# Autodesk Inventor assembly: Estructura Lámina
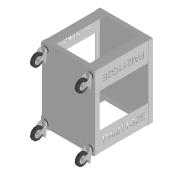
[picture p0: Inventor's stored thumbnail of the model, 180x180]
Saved by Autodesk Inventor 2021 (Build 250183000, 183)
## iProperties
Created: 2021-04-18
Part Number: Estructura Lámina
Document SubType Name: Assembly
Designer: carlo
Author: carlo
## Documents named in this file (4)
- C:\Users\carlo\Desktop\Concepto\Estructura laminas\Estructura Lámina.iam
- C:\Users\carlo\Desktop\Concepto\Estructura laminas\Laterales.ipt
- C:\Users\carlo\Desktop\Concepto\Estructura laminas\Tapa.ipt
- C:\Users\carlo\Desktop\Concepto\Estructura laminas\CASTER_WHEEL_FREE_Ø125mm.iam
## Components (10 placed, 3 different names)
1. Laterales:1 — Coincidencia:1, Coincidencia:2, Coincidencia:3
2. Tapa:1 — Coincidencia:1, Coincidencia:2, Coincidencia:3, Coincidencia:4, Coincidencia:5, Coincidencia:6, Coincidencia:7, Coincidencia:8, Coincidencia:9, Coincidencia:10, Coincidencia:11, Coincidencia:12
3. Laterales:2 — Coincidencia:7, Coincidencia:8, Coincidencia:9, Coincidencia:13, Coincidencia:14, Coincidencia:15
4. Laterales:3 — Coincidencia:10, Coincidencia:11, Coincidencia:12
5. Laterales:4 — Coincidencia:4, Coincidencia:5, Coincidencia:6
6. Tapa:2 — Coincidencia:13, Coincidencia:14, Coincidencia:15, Coincidencia:16, Nivelación:1, Nivelación:2, Coincidencia:17, Nivelación:3, Nivelación:4, Coincidencia:18, Nivelación:5, Nivelación:6, Coincidencia:19, Nivelación:7, Nivelación:8
7. CASTER_WHEEL_FREE_Ø125mm:1 [sub-assembly] — Coincidencia:16, Nivelación:1, Nivelación:2
8. CASTER_WHEEL_FREE_Ø125mm:2 [sub-assembly] — Coincidencia:19, Nivelación:7, Nivelación:8
9. CASTER_WHEEL_FREE_Ø125mm:3 [sub-assembly] — Coincidencia:18, Nivelación:5, Nivelación:6
10. CASTER_WHEEL_FREE_Ø125mm:4 [sub-assembly] — Coincidencia:17, Nivelación:3, Nivelación:4
## Relationships (27: Mate 19, Flush 8)
- Coincidencia:1 [Mate]: Laterales:1 ↔ Tapa:1
- Coincidencia:2 [Mate]: Laterales:1 ↔ Tapa:1
- Coincidencia:3 [Mate]: Laterales:1 ↔ Tapa:1
- Coincidencia:4 [Mate]: Tapa:1 ↔ Laterales:4
- Coincidencia:5 [Mate]: Tapa:1 ↔ Laterales:4
- Coincidencia:6 [Mate]: Tapa:1 ↔ Laterales:4
- Coincidencia:7 [Mate]: Tapa:1 ↔ Laterales:2
- Coincidencia:8 [Mate]: Tapa:1 ↔ Laterales:2
- Coincidencia:9 [Mate]: Tapa:1 ↔ Laterales:2
- Coincidencia:10 [Mate]: Tapa:1 ↔ Laterales:3
- Coincidencia:11 [Mate]: Tapa:1 ↔ Laterales:3
- Coincidencia:12 [Mate]: Tapa:1 ↔ Laterales:3
- Coincidencia:13 [Mate]: Laterales:2 ↔ Tapa:2
- Coincidencia:14 [Mate]: Laterales:2 ↔ Tapa:2
- Coincidencia:15 [Mate]: Laterales:2 ↔ Tapa:2
- Coincidencia:16 [Mate]: Tapa:2 ↔ CASTER_WHEEL_FREE_Ø125mm:1
- Nivelación:1 [Flush]: Tapa:2 ↔ CASTER_WHEEL_FREE_Ø125mm:1
- Nivelación:2 [Flush]: Tapa:2 ↔ CASTER_WHEEL_FREE_Ø125mm:1
- Coincidencia:17 [Mate]: Tapa:2 ↔ CASTER_WHEEL_FREE_Ø125mm:4
- Nivelación:3 [Flush]: Tapa:2 ↔ CASTER_WHEEL_FREE_Ø125mm:4
- Nivelación:4 [Flush]: Tapa:2 ↔ CASTER_WHEEL_FREE_Ø125mm:4
- Coincidencia:18 [Mate]: Tapa:2 ↔ CASTER_WHEEL_FREE_Ø125mm:3
- Nivelación:5 [Flush]: Tapa:2 ↔ CASTER_WHEEL_FREE_Ø125mm:3
- Nivelación:6 [Flush]: Tapa:2 ↔ CASTER_WHEEL_FREE_Ø125mm:3
- Coincidencia:19 [Mate]: Tapa:2 ↔ CASTER_WHEEL_FREE_Ø125mm:2
- Nivelación:7 [Flush]: Tapa:2 ↔ CASTER_WHEEL_FREE_Ø125mm:2
- Nivelación:8 [Flush]: Tapa:2 ↔ CASTER_WHEEL_FREE_Ø125mm:2
